# Autodesk Inventor assembly: ONDERPLAAT
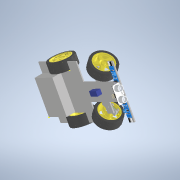
[picture p0: Inventor's stored thumbnail of the model, 180x180]
Saved by Autodesk Inventor 2022 (Build 260153000, 153)
## iProperties
Created: 2021-12-16
Part Number: ONDERPLAAT
Document SubType Name: Assembly
Designer: keemi
Author: keemi
## Documents named in this file (9)
- C:\Users\keemi\OneDrive\Bureaublad\repo's\projecten\Auto\modellen\inventor\auto moddel\ONDERPLAAT.iam
- C:\Users\keemi\OneDrive\Bureaublad\repo's\projecten\Auto\modellen\inventor\auto moddel\onderkant.ipt
- C:\Users\keemi\OneDrive\Bureaublad\repo's\projecten\Auto\modellen\inventor\geared-dc-motor-for-arduino-applications-1.snapshot.2\Hobi - Motor DC 1.ipt
- C:\Users\keemi\OneDrive\Bureaublad\repo's\projecten\Auto\modellen\inventor\wheel-arduino-1.snapshot.2\Wheel ALL.ipt
- C:\Users\keemi\OneDrive\Bureaublad\repo's\projecten\Auto\modellen\inventor\SG90\SG90 v1.ipt
- C:\Users\keemi\OneDrive\Bureaublad\repo's\projecten\Auto\modellen\inventor\auto moddel\STUURAS.ipt
- C:\Users\keemi\OneDrive\Bureaublad\repo's\projecten\Auto\modellen\inventor\ir_sensor-1.snapshot.1\IR sensor.ipt
- C:\Users\keemi\OneDrive\Bureaublad\repo's\projecten\Auto\modellen\inventor\ultrasonic-sensor-hc-sr04-4.snapshot.11\Ultrasonic Sensor HC-SR04\Ultrasonic Sensor HC-SR04.ipt
- C:\Users\keemi\OneDrive\Bureaublad\repo's\projecten\Auto\modellen\inventor\POWERBANK.ipt
## Components (14 placed, 8 different names)
1. onderkant:1 — Mate:9, Flush:1, Mate:10, Flush:3, Flush:4, Mate:11, Flush:5, Flush:6, Mate:16, Mate:18, Mate:19, Mate:21, Mate:22, Flush:8, Flush:9, Mate:23, Flush:10, Flush:11, Mate:24, Mate:25, Angle:1, Angle:2, Mate:26, Flush:12
2. Hobi - Motor DC 1:1 — Mate:1, Mate:2, Mate:10, Flush:2, Flush:4
3. Wheel ALL:1 — Mate:1, Mate:2
4. Hobi - Motor DC 1:2 — Mate:9, Flush:1, Flush:2, Flush:3
5. Wheel ALL:2
6. SG90 v1:1 — Mate:11, Flush:5, Flush:6
7. STUURAS:1 — Mate:12, Mate:13, Mate:16, Mate:18, Angle:2
8. Wheel ALL:3 — Mate:12, Mate:13
9. STUURAS:2 — Mate:19, Mate:21, Angle:1
10. Wheel ALL:4
11. IR sensor:1 — Mate:22, Flush:8, Flush:9
12. Ultrasonic Sensor HC-SR04:1 — Mate:23, Flush:10
13. IR sensor:2 — Flush:11, Mate:24, Mate:25
14. POWERBANK:1 — Mate:26, Flush:12
## Relationships (33: Mate 20, Flush 11, Angle 2)
- Mate:1: Hobi - Motor DC 1:1 ↔ Wheel ALL:1
- Mate:2: Hobi - Motor DC 1:1 ↔ Wheel ALL:1
- [Mate]: Hobi - Motor DC 1:2 ↔ Wheel ALL:2
- [Mate]: Hobi - Motor DC 1:2 ↔ Wheel ALL:2
- Mate:9: onderkant:1 ↔ Hobi - Motor DC 1:2
- Flush:1 (60 mm): onderkant:1 ↔ Hobi - Motor DC 1:2
- Mate:10: onderkant:1 ↔ Hobi - Motor DC 1:1
- Flush:2: Hobi - Motor DC 1:1 ↔ Hobi - Motor DC 1:2
- Flush:3 (26 mm): onderkant:1 ↔ Hobi - Motor DC 1:2
- Flush:4 (26 mm): onderkant:1 ↔ Hobi - Motor DC 1:1
- Mate:11: onderkant:1 ↔ SG90 v1:1
- Flush:5 (70 mm): onderkant:1 ↔ SG90 v1:1
- Flush:6 (65 mm): onderkant:1 ↔ SG90 v1:1
- Mate:12: STUURAS:1 ↔ Wheel ALL:3
- Mate:13: STUURAS:1 ↔ Wheel ALL:3
- [Mate]: STUURAS:2 ↔ Wheel ALL:4
- [Mate]: STUURAS:2 ↔ Wheel ALL:4
- Mate:16: onderkant:1 ↔ STUURAS:1
- Mate:18: onderkant:1 ↔ STUURAS:1
- Mate:19: onderkant:1 ↔ STUURAS:2
- Mate:21: onderkant:1 ↔ STUURAS:2
- Mate:22: onderkant:1 ↔ IR sensor:1
- Flush:8 (3 mm): onderkant:1 ↔ IR sensor:1
- Flush:9: onderkant:1 ↔ IR sensor:1
- Mate:23: onderkant:1 ↔ Ultrasonic Sensor HC-SR04:1
- Flush:10 (3 mm): onderkant:1 ↔ Ultrasonic Sensor HC-SR04:1
- Flush:11 (3 mm): onderkant:1 ↔ IR sensor:2
- Mate:24: onderkant:1 ↔ IR sensor:2
- Mate:25: onderkant:1 ↔ IR sensor:2
- Angle:1 (315 deg): onderkant:1 ↔ STUURAS:2
- Angle:2 (45 deg): onderkant:1 ↔ STUURAS:1
- Mate:26: onderkant:1 ↔ POWERBANK:1
- Flush:12 (3 mm): onderkant:1 ↔ POWERBANK:1
## Named parameters: d2_d0 = 0 mm, d3_d1 = 0 mm, d24_d22 = 0 mm, d25_d23 = 0 mm
